# Autodesk Inventor assembly: Placa y Base
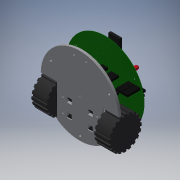
[picture p0: Inventor's stored thumbnail of the model, 180x180]
Saved by Autodesk Inventor 2017 (Build 210142000, 142)
## iProperties
Part Number: Placa y Base
Material: Genérico
Document SubType Name: Assembly
Designer: fam
Author: fam
## Documents named in this file (4)
- C:\Users\fam\Desktop\UVG\Ciclo 9\Megaproyecto\Megaproyecto\Diseños Inventor Fase 2\Placa y Base.iam
- C:\Users\fam\Desktop\UVG\Ciclo 9\Megaproyecto\Megaproyecto\Diseños Inventor Fase 2\Base.ipt
- C:\Users\fam\Desktop\UVG\Ciclo 9\Megaproyecto\Megaproyecto\Diseños Inventor Fase 2\Encoder-Motor-Llanta.iam
- C:\Users\fam\Desktop\UVG\Ciclo 9\Megaproyecto\Megaproyecto\Diseños Inventor Fase 2\PCB.iam
## Components (4 placed, 3 different names)
1. Base:1 — Coincidencia:1, Coincidencia:2, Coincidencia:3, Coincidencia:4, Coincidencia:5, Coincidencia:6, Coincidencia:7, Coincidencia:8, Nivelación:1
2. Encoder-Motor-Llanta:1 [sub-assembly] — Coincidencia:1, Coincidencia:2, Coincidencia:3
3. Encoder-Motor-Llanta:2 [sub-assembly] — Coincidencia:4, Coincidencia:5, Coincidencia:6
4. PCB:1 [sub-assembly] — Coincidencia:7, Coincidencia:8, Nivelación:1
## Relationships (9: Mate 8, Flush 1)
- Coincidencia:1 [Mate]: Base:1 ↔ Encoder-Motor-Llanta:1
- Coincidencia:2 [Mate]: Base:1 ↔ Encoder-Motor-Llanta:1
- Coincidencia:3 [Mate]: Base:1 ↔ Encoder-Motor-Llanta:1
- Coincidencia:4 [Mate]: Base:1 ↔ Encoder-Motor-Llanta:2
- Coincidencia:5 [Mate]: Base:1 ↔ Encoder-Motor-Llanta:2
- Coincidencia:6 [Mate]: Base:1 ↔ Encoder-Motor-Llanta:2
- Coincidencia:7 [Mate]: Base:1 ↔ PCB:1
- Coincidencia:8 [Mate]: Base:1 ↔ PCB:1
- Nivelación:1 [Flush] (-30 mm): Base:1 ↔ PCB:1
